# Autodesk Inventor assembly: 201
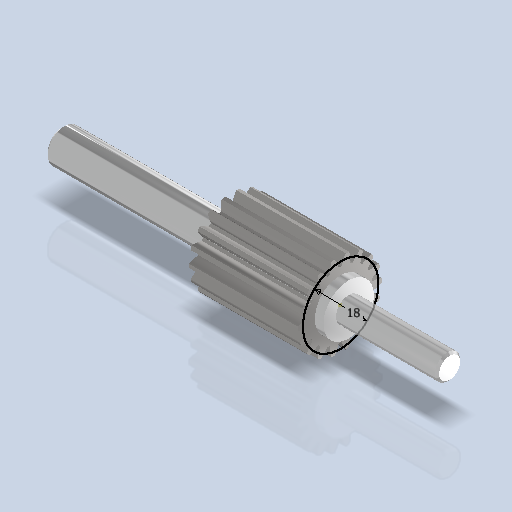
[picture p0: Inventor's stored thumbnail of the model, 512x512]
Saved by Autodesk Inventor 2024 (Build 280153000, 153)
## iProperties
Created: 2024-07-12
Part Number: 201
Document SubType Name: Assembly
Designer: ffogue
Author: ffogue
## Documents named in this file (3)
- C:\Users\ffogue\OneDrive - MuM - OM\Dokumente\Inventor\GearBox\201.iam
- C:\Users\ffogue\OneDrive - MuM - OM\Dokumente\Inventor\GearBox\201 Welle.ipt
- C:\Users\ffogue\OneDrive - MuM - OM\Dokumente\Inventor\GearBox\201_gear.iam
## Components (2 placed, 2 different names)
1. 201 Welle:1 — Einfügen:1
2. 201_gear:1 [sub-assembly] — Einfügen:1
## Relationships (1: Insert 1)
- Einfügen:1 [Insert] (-28 mm): 201 Welle:1 ↔ 201_gear:1
